# Autodesk Inventor assembly: MechanumChassis
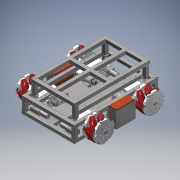
[picture p0: Inventor's stored thumbnail of the model, 180x180]
Saved by Autodesk Inventor 2018 (Build 220112000, 112)
## iProperties
Created: 2017-10-18
Part Number: MechanumChassis
Document SubType Name: Weldment
Designer: Bryce Richards
Mass: 42172.1 g
Surface Area: 44852.8 cm^2
Volume: 5448.29 cm^3
Density: 7.74044 g/cm^3
Weld Material: Steel, Mild, Welded
Author: Bryce Richards
## Documents named in this file (20)
- C:\Users\P136265\Documents\GitHub\mecanum-cad\MechanumChassis.iam
- C:\Users\P136265\Documents\GitHub\mecanum-cad\MecanumFrame2.iam
- C:\Users\P136265\Documents\GitHub\mecanum-cad\WheelShaft.ipt
- C:\Users\P136265\Documents\GitHub\mecanum-cad\Mecanum_Assembly.iam
- C:\Users\P136265\Documents\Inventor\Content Center Files\R2018\en-US\AS 1112 (2)\AS 1112 - M4  Type 5.ipt
- C:\Users\P136265\Documents\GitHub\mecanum-cad\LiftBase.ipt
- C:\Users\P136265\Documents\GitHub\mecanum-cad\BatteryBox_NP1812.ipt
- C:\Users\P136265\Documents\GitHub\mecanum-cad\NP18-12 Battery.ipt
- C:\Users\P136265\Documents\GitHub\mecanum-cad\BearingHousing.iam
- C:\Users\P136265\Documents\Inventor\Content Center Files\R2018\en-US\AS 1110\AS 1110 - M8 x 50.ipt
- C:\Users\P136265\Documents\GitHub\mecanum-cad\mount.ipt
- C:\Users\P136265\Documents\GitHub\mecanum-cad\Nema 23 Stepper Motor Bipolar L=56mm w Gear Ratio 41 Planetary Gearbox.ipt
- C:\Users\P136265\Documents\GitHub\mecanum-cad\LiftAssembly_Through.iam
- C:\Users\P136265\Documents\Inventor\Content Center Files\R2018\en-US\BS EN 24035\ISO 4035 - M20BS EN.ipt
- C:\Users\P136265\Documents\Inventor\Content Center Files\R2018\en-US\AS 1420\AS 1420 - 1973 - M4 x 12.ipt
- C:\Users\P136265\Documents\Inventor\Content Center Files\R2018\en-US\AS 1112 (2)\AS 1112 - M8  Type 8.ipt
- C:\Users\P136265\Documents\GitHub\mecanum-cad\SyncHub_Assembly.iam
- C:\Users\P136265\Documents\Inventor\Content Center Files\R2018\en-US\BS EN 24035\ISO 4035 - M12BS EN.ipt
- C:\Users\P136265\Documents\GitHub\mecanum-cad\LiftPlate.iam
- C:\Users\P136265\Documents\mecanum-cad\MechanumChassis\AIP\FEA\cayefugld.fres
## Components (91 placed, 18 different names)
1. MecanumFrame2:1 [sub-assembly] — Mate:90, Angle:5, Angle:6, Angle:7, Mate:386, Flush:32, Flush:33, Mate:486, Mate:487, Mate:488, Mate:489, Mate:494, Mate:500, Mate:501, Mate:502, Mate:503, Mate:504, Mate:594, Angle:41, Mate:607, Mate:608, Mate:641, Mate:642, Mate:643, Mate:644, Mate:645, Mate:646, Angle:49, Angle:51, Insert:1, Insert:2, Insert:3, Insert:4, Insert:5, Insert:6, Insert:7, Insert:8, Insert:9, Insert:10, Insert:11, Insert:12, Insert:13, Insert:14, Insert:15, Insert:16, Angle:52, Angle:53
2. Mecanum_Assembly:1 [sub-assembly] — Mate:617, Mate:618, Angle:44, Mate:654
3. Mecanum_Assembly:2 [sub-assembly] — Mate:613, Mate:614, Angle:43, Mate:652
4. Mecanum_Assembly:3 [sub-assembly] — Mate:621, Mate:622, Mate:650
5. Mecanum_Assembly:4 [sub-assembly] — Mate:609, Mate:610, Angle:42, Mate:648
6. LiftBase:1 — Mate:386, Flush:32, Flush:33, Mate:606, Mate:635, Mate:637, Mate:639
7. BatteryBox_NP1812:1 — Mate:459, Mate:461
8. BatteryBox_NP1812:2 — Mate:462, Mate:464
9. NP18-12 Battery:1 — Mate:459, Mate:461, Angle:45, Angle:46
10. NP18-12 Battery:2 — Mate:462, Mate:464, Angle:40, Angle:47
11. AS 1112 (2) - Metric M4  Type 5:17
12. AS 1112 (2) - Metric M4  Type 5:18
13. AS 1112 (2) - Metric M4  Type 5:19
14. AS 1112 (2) - Metric M4  Type 5:20
15. AS 1112 (2) - Metric M4  Type 5:21
16. AS 1112 (2) - Metric M4  Type 5:22
17. AS 1112 (2) - Metric M4  Type 5:23
18. AS 1112 (2) - Metric M4  Type 5:24
19. BearingHousing:1 [sub-assembly] — Mate:486, Mate:487, Mate:488, Mate:489, Mate:493, Mate:611, Mate:612, Mate:660, Mate:672, Mate:674, Mate:676, Mate:678
20. BearingHousing:2 [sub-assembly] — Mate:493, Mate:494, Mate:594, Mate:615, Mate:616, Mate:658, Mate:696, Mate:698, Mate:700, Mate:702
21. BearingHousing:3 [sub-assembly] — Mate:503, Mate:504, Mate:623, Mate:624, Mate:662, Mate:680, Mate:682, Mate:684, Mate:686
22. BearingHousing:4 [sub-assembly] — Mate:500, Mate:501, Mate:502, Mate:619, Mate:620, Mate:656, Mate:688, Mate:690, Mate:692, Mate:694
23. mount:1 — Mate:603, Mate:604, Mate:605, Mate:606
24. Nema 23 Stepper Motor Bipolar L=56mm w Gear Ratio 41 Planetary Gearbox:1 — Mate:603, Mate:604, Mate:605, Angle:40, Angle:41, Flush:34, Mate:625, Mate:711
25. LiftAssembly_Through:1 [sub-assembly] — Mate:607, Mate:608, Angle:48
26. WheelShaft:1 — Mate:621, Mate:622, Mate:623, Mate:624, Flush:37, Mate:640, Mate:649, Mate:661, Mate:709, Flush:38, Mate:715
27. WheelShaft:2 — Mate:617, Mate:618, Mate:619, Mate:620, Angle:44, Flush:36, Mate:638, Mate:653, Mate:655, Mate:708, Mate:713
28. WheelShaft:3 — Mate:613, Mate:614, Mate:615, Mate:616, Angle:43, Flush:35, Mate:636, Mate:651, Mate:657, Mate:704, Mate:717
29. WheelShaft:4 — Mate:609, Mate:610, Angle:42, Mate:611, Mate:612, Flush:34, Mate:625, Mate:647, Mate:659, Mate:712, Flush:39, Mate:719
30. mount:2 — Mate:626, Mate:627, Mate:628, Mate:637
31. mount:3 — Mate:629, Mate:630, Mate:631, Mate:639
32. mount:4 — Mate:632, Mate:633, Mate:634, Mate:635
33. Nema 23 Stepper Motor Bipolar L=56mm w Gear Ratio 41 Planetary Gearbox:2 — Mate:626, Mate:627, Mate:628, Angle:46, Flush:36, Mate:638, Mate:706
34. Nema 23 Stepper Motor Bipolar L=56mm w Gear Ratio 41 Planetary Gearbox:3 — Mate:629, Mate:630, Mate:631, Angle:47, Flush:37, Mate:640, Mate:710
35. Nema 23 Stepper Motor Bipolar L=56mm w Gear Ratio 41 Planetary Gearbox:4 — Mate:632, Mate:633, Mate:634, Angle:45, Flush:35, Mate:636, Mate:705
36. LiftAssembly_Through:2 [sub-assembly] — Mate:641, Mate:642, Angle:50, Angle:51, Mate:663, Mate:664, Mate:665, Mate:666, Mate:667, Mate:668, Mate:669, Mate:670
37. LiftAssembly_Through:3 [sub-assembly] — Mate:643, Mate:644, Angle:50, Mate:721
38. LiftAssembly_Through:4 [sub-assembly] — Mate:645, Mate:646, Angle:48, Angle:49
39. BS EN 24035 - Metric M20:1 — Mate:647, Mate:648
40. BS EN 24035 - Metric M20:2 — Mate:649, Mate:650
41. BS EN 24035 - Metric M20:3 — Mate:651, Mate:652
42. BS EN 24035 - Metric M20:4 — Mate:653, Mate:654
43. BS EN 24035 - Metric M20:5 — Mate:655, Mate:656, Mate:707
44. BS EN 24035 - Metric M20:6 — Mate:657, Mate:658, Mate:703
45. BS EN 24035 - Metric M20:7 — Mate:659, Mate:660
46. BS EN 24035 - Metric M20:8 — Mate:661, Mate:662
47. AS 1110 - Metric M8 x 50:1 — Insert:1, Mate:697
48. AS 1110 - Metric M8 x 50:2 — Insert:2, Mate:699
49. AS 1110 - Metric M8 x 50:3 — Insert:3, Mate:693
50. AS 1110 - Metric M8 x 50:4 — Insert:4, Mate:691
51. AS 1110 - Metric M8 x 50:5 — Insert:5, Mate:695
52. AS 1110 - Metric M8 x 50:6 — Insert:6, Mate:701
53. AS 1110 - Metric M8 x 50:7 — Insert:7, Mate:687
54. AS 1110 - Metric M8 x 50:8 — Insert:8, Mate:689
55. AS 1110 - Metric M8 x 50:9 — Insert:9, Mate:675
56. AS 1110 - Metric M8 x 50:10 — Insert:10, Mate:677
57. AS 1110 - Metric M8 x 50:11 — Insert:11, Mate:685
58. AS 1110 - Metric M8 x 50:12 — Insert:12, Mate:683
59. AS 1110 - Metric M8 x 50:13 — Insert:13, Mate:671
60. AS 1110 - Metric M8 x 50:14 — Insert:14, Mate:673
61. AS 1110 - Metric M8 x 50:15 — Insert:15, Mate:679
62. AS 1110 - Metric M8 x 50:16 — Insert:16, Mate:681
63. AS 1420 - Metric M4 x 12:1 — Mate:663, Mate:664
64. AS 1420 - Metric M4 x 12:2 — Mate:665, Mate:666
65. AS 1420 - Metric M4 x 12:3 — Mate:667, Mate:668
66. AS 1420 - Metric M4 x 12:4 — Mate:669, Mate:670
67. AS 1112 (2) - Metric M8  Type 8:1 — Mate:671, Mate:672
68. AS 1112 (2) - Metric M8  Type 8:2 — Mate:673, Mate:674
69. AS 1112 (2) - Metric M8  Type 8:3 — Mate:675, Mate:676
70. AS 1112 (2) - Metric M8  Type 8:4 — Mate:677, Mate:678
71. AS 1112 (2) - Metric M8  Type 8:5 — Mate:679, Mate:680
72. AS 1112 (2) - Metric M8  Type 8:6 — Mate:681, Mate:682
73. AS 1112 (2) - Metric M8  Type 8:7 — Mate:683, Mate:684
74. AS 1112 (2) - Metric M8  Type 8:8 — Mate:685, Mate:686
75. AS 1112 (2) - Metric M8  Type 8:9 — Mate:687, Mate:688
76. AS 1112 (2) - Metric M8  Type 8:10 — Mate:689, Mate:690
77. AS 1112 (2) - Metric M8  Type 8:11 — Mate:691, Mate:692
78. AS 1112 (2) - Metric M8  Type 8:12 — Mate:693, Mate:694
79. AS 1112 (2) - Metric M8  Type 8:13 — Mate:695, Mate:696
80. AS 1112 (2) - Metric M8  Type 8:14 — Mate:697, Mate:698
81. AS 1112 (2) - Metric M8  Type 8:15 — Mate:699, Mate:700
82. AS 1112 (2) - Metric M8  Type 8:16 — Mate:701, Mate:702
83. SyncHub_Assembly:1 [sub-assembly] — Mate:703, Mate:704, Mate:705, Mate:718
84. SyncHub_Assembly:2 [sub-assembly] — Mate:711, Mate:712, Flush:39, Mate:720
85. SyncHub_Assembly:3 [sub-assembly] — Mate:706, Mate:707, Mate:708, Mate:714
86. SyncHub_Assembly:4 [sub-assembly] — Mate:709, Mate:710, Flush:38, Mate:716
87. BS EN 24035 - Metric M12:1 — Mate:713, Mate:714
88. BS EN 24035 - Metric M12:2 — Mate:715, Mate:716
89. BS EN 24035 - Metric M12:3 — Mate:717, Mate:718
90. BS EN 24035 - Metric M12:4 — Mate:719, Mate:720
91. LiftPlate:1 [sub-assembly] — Angle:52, Angle:53, Mate:721
## Relationships (178: Mate 137, Angle 17, Insert 16, Flush 8)
- Mate:90: MecanumFrame2:1
- Angle:5 (0 deg): MecanumFrame2:1
- Angle:6 (0 deg): MecanumFrame2:1
- Angle:7 (0 deg): MecanumFrame2:1
- Mate:386: MecanumFrame2:1 ↔ LiftBase:1
- Flush:32 (2.5 mm): MecanumFrame2:1 ↔ LiftBase:1
- Flush:33 (2.5 mm): MecanumFrame2:1 ↔ LiftBase:1
- Mate:459: BatteryBox_NP1812:1 ↔ NP18-12 Battery:1
- Mate:461 (2 mm): BatteryBox_NP1812:1 ↔ NP18-12 Battery:1
- Mate:462: BatteryBox_NP1812:2 ↔ NP18-12 Battery:2
- Mate:464 (2 mm): BatteryBox_NP1812:2 ↔ NP18-12 Battery:2
- Mate:486: MecanumFrame2:1 ↔ BearingHousing:1
- Mate:487: MecanumFrame2:1 ↔ BearingHousing:1
- Mate:488: MecanumFrame2:1 ↔ BearingHousing:1
- Mate:489: MecanumFrame2:1 ↔ BearingHousing:1
- Mate:493: BearingHousing:1 ↔ BearingHousing:2
- Mate:494: MecanumFrame2:1 ↔ BearingHousing:2
- Mate:500: MecanumFrame2:1 ↔ BearingHousing:4
- Mate:501: MecanumFrame2:1 ↔ BearingHousing:4
- Mate:502: MecanumFrame2:1 ↔ BearingHousing:4
- Mate:503: MecanumFrame2:1 ↔ BearingHousing:3
- Mate:504: MecanumFrame2:1 ↔ BearingHousing:3
- Mate:594: MecanumFrame2:1 ↔ BearingHousing:2
- Mate:603: mount:1 ↔ Nema 23 Stepper Motor Bipolar L=56mm w Gear Ratio 41 Planetary Gearbox:1
- Mate:604: mount:1 ↔ Nema 23 Stepper Motor Bipolar L=56mm w Gear Ratio 41 Planetary Gearbox:1
- Mate:605: mount:1 ↔ Nema 23 Stepper Motor Bipolar L=56mm w Gear Ratio 41 Planetary Gearbox:1
- Mate:606: LiftBase:1 ↔ mount:1
- Angle:40 (180 deg): NP18-12 Battery:2 ↔ Nema 23 Stepper Motor Bipolar L=56mm w Gear Ratio 41 Planetary Gearbox:1
- Angle:41 (0 deg): MecanumFrame2:1 ↔ Nema 23 Stepper Motor Bipolar L=56mm w Gear Ratio 41 Planetary Gearbox:1
- Mate:607: MecanumFrame2:1 ↔ LiftAssembly_Through:1
- Mate:608: MecanumFrame2:1 ↔ LiftAssembly_Through:1
- Mate:609: Mecanum_Assembly:4 ↔ WheelShaft:4
- Mate:610: Mecanum_Assembly:4 ↔ WheelShaft:4
- Angle:42 (0 deg): Mecanum_Assembly:4 ↔ WheelShaft:4
- Mate:611: BearingHousing:1 ↔ WheelShaft:4
- Mate:612: BearingHousing:1 ↔ WheelShaft:4
- Flush:34 (10 mm): Nema 23 Stepper Motor Bipolar L=56mm w Gear Ratio 41 Planetary Gearbox:1 ↔ WheelShaft:4
- Mate:613: Mecanum_Assembly:2 ↔ WheelShaft:3
- Mate:614: Mecanum_Assembly:2 ↔ WheelShaft:3
- Mate:615: BearingHousing:2 ↔ WheelShaft:3
- Mate:616: BearingHousing:2 ↔ WheelShaft:3
- Angle:43 (0 deg): Mecanum_Assembly:2 ↔ WheelShaft:3
- Mate:617: Mecanum_Assembly:1 ↔ WheelShaft:2
- Mate:618: Mecanum_Assembly:1 ↔ WheelShaft:2
- Mate:619: BearingHousing:4 ↔ WheelShaft:2
- Mate:620: BearingHousing:4 ↔ WheelShaft:2
- Angle:44 (0 deg): Mecanum_Assembly:1 ↔ WheelShaft:2
- Mate:621: Mecanum_Assembly:3 ↔ WheelShaft:1
- Mate:622: Mecanum_Assembly:3 ↔ WheelShaft:1
- Mate:623: BearingHousing:3 ↔ WheelShaft:1
- Mate:624: BearingHousing:3 ↔ WheelShaft:1
- Mate:625 (107.5 mm): Nema 23 Stepper Motor Bipolar L=56mm w Gear Ratio 41 Planetary Gearbox:1 ↔ WheelShaft:4
- Mate:626: mount:2 ↔ Nema 23 Stepper Motor Bipolar L=56mm w Gear Ratio 41 Planetary Gearbox:2
- Mate:627: mount:2 ↔ Nema 23 Stepper Motor Bipolar L=56mm w Gear Ratio 41 Planetary Gearbox:2
- Mate:628: mount:2 ↔ Nema 23 Stepper Motor Bipolar L=56mm w Gear Ratio 41 Planetary Gearbox:2
- Mate:629: mount:3 ↔ Nema 23 Stepper Motor Bipolar L=56mm w Gear Ratio 41 Planetary Gearbox:3
- Mate:630: mount:3 ↔ Nema 23 Stepper Motor Bipolar L=56mm w Gear Ratio 41 Planetary Gearbox:3
- Mate:631: mount:3 ↔ Nema 23 Stepper Motor Bipolar L=56mm w Gear Ratio 41 Planetary Gearbox:3
- Mate:632: mount:4 ↔ Nema 23 Stepper Motor Bipolar L=56mm w Gear Ratio 41 Planetary Gearbox:4
- Mate:633: mount:4 ↔ Nema 23 Stepper Motor Bipolar L=56mm w Gear Ratio 41 Planetary Gearbox:4
- Mate:634: mount:4 ↔ Nema 23 Stepper Motor Bipolar L=56mm w Gear Ratio 41 Planetary Gearbox:4
- Mate:635: LiftBase:1 ↔ mount:4
- Angle:45 (0 deg): NP18-12 Battery:1 ↔ Nema 23 Stepper Motor Bipolar L=56mm w Gear Ratio 41 Planetary Gearbox:4
- Flush:35 (10 mm): WheelShaft:3 ↔ Nema 23 Stepper Motor Bipolar L=56mm w Gear Ratio 41 Planetary Gearbox:4
- Mate:636 (107.5 mm): WheelShaft:3 ↔ Nema 23 Stepper Motor Bipolar L=56mm w Gear Ratio 41 Planetary Gearbox:4
- Mate:637: LiftBase:1 ↔ mount:2
- Angle:46 (0 deg): NP18-12 Battery:1 ↔ Nema 23 Stepper Motor Bipolar L=56mm w Gear Ratio 41 Planetary Gearbox:2
- Flush:36 (10 mm): WheelShaft:2 ↔ Nema 23 Stepper Motor Bipolar L=56mm w Gear Ratio 41 Planetary Gearbox:2
- Mate:638 (107.5 mm): WheelShaft:2 ↔ Nema 23 Stepper Motor Bipolar L=56mm w Gear Ratio 41 Planetary Gearbox:2
- Angle:47 (0 deg): NP18-12 Battery:2 ↔ Nema 23 Stepper Motor Bipolar L=56mm w Gear Ratio 41 Planetary Gearbox:3
- Mate:639: LiftBase:1 ↔ mount:3
- Flush:37 (10 mm): WheelShaft:1 ↔ Nema 23 Stepper Motor Bipolar L=56mm w Gear Ratio 41 Planetary Gearbox:3
- Mate:640 (107.5 mm): WheelShaft:1 ↔ Nema 23 Stepper Motor Bipolar L=56mm w Gear Ratio 41 Planetary Gearbox:3
- Mate:641: MecanumFrame2:1 ↔ LiftAssembly_Through:2
- Mate:642: MecanumFrame2:1 ↔ LiftAssembly_Through:2
- Mate:643: MecanumFrame2:1 ↔ LiftAssembly_Through:3
- Mate:644: MecanumFrame2:1 ↔ LiftAssembly_Through:3
- Mate:645: MecanumFrame2:1 ↔ LiftAssembly_Through:4
- Mate:646: MecanumFrame2:1 ↔ LiftAssembly_Through:4
- Angle:48 (0 deg): LiftAssembly_Through:1 ↔ LiftAssembly_Through:4
- Angle:49 (0 deg): MecanumFrame2:1 ↔ LiftAssembly_Through:4
- Angle:50 (0 deg): LiftAssembly_Through:2 ↔ LiftAssembly_Through:3
- Angle:51 (0 deg): MecanumFrame2:1 ↔ LiftAssembly_Through:2
- Mate:647: WheelShaft:4 ↔ BS EN 24035 - Metric M20:1
- Mate:648: Mecanum_Assembly:4 ↔ BS EN 24035 - Metric M20:1
- Mate:649: WheelShaft:1 ↔ BS EN 24035 - Metric M20:2
- Mate:650: Mecanum_Assembly:3 ↔ BS EN 24035 - Metric M20:2
- Mate:651: WheelShaft:3 ↔ BS EN 24035 - Metric M20:3
- Mate:652: Mecanum_Assembly:2 ↔ BS EN 24035 - Metric M20:3
- Mate:653: WheelShaft:2 ↔ BS EN 24035 - Metric M20:4
- Mate:654: Mecanum_Assembly:1 ↔ BS EN 24035 - Metric M20:4
- Mate:655: WheelShaft:2 ↔ BS EN 24035 - Metric M20:5
- Mate:656: BearingHousing:4 ↔ BS EN 24035 - Metric M20:5
- Mate:657: WheelShaft:3 ↔ BS EN 24035 - Metric M20:6
- Mate:658: BearingHousing:2 ↔ BS EN 24035 - Metric M20:6
- Mate:659: WheelShaft:4 ↔ BS EN 24035 - Metric M20:7
- Mate:660: BearingHousing:1 ↔ BS EN 24035 - Metric M20:7
- Mate:661: WheelShaft:1 ↔ BS EN 24035 - Metric M20:8
- Mate:662: BearingHousing:3 ↔ BS EN 24035 - Metric M20:8
- Insert:1: MecanumFrame2:1 ↔ AS 1110 - Metric M8 x 50:1
- Insert:2: MecanumFrame2:1 ↔ AS 1110 - Metric M8 x 50:2
- Insert:3: MecanumFrame2:1 ↔ AS 1110 - Metric M8 x 50:3
- Insert:4: MecanumFrame2:1 ↔ AS 1110 - Metric M8 x 50:4
- Insert:5: MecanumFrame2:1 ↔ AS 1110 - Metric M8 x 50:5
- Insert:6: MecanumFrame2:1 ↔ AS 1110 - Metric M8 x 50:6
- Insert:7: MecanumFrame2:1 ↔ AS 1110 - Metric M8 x 50:7
- Insert:8: MecanumFrame2:1 ↔ AS 1110 - Metric M8 x 50:8
- Insert:9: MecanumFrame2:1 ↔ AS 1110 - Metric M8 x 50:9
- Insert:10: MecanumFrame2:1 ↔ AS 1110 - Metric M8 x 50:10
- Insert:11: MecanumFrame2:1 ↔ AS 1110 - Metric M8 x 50:11
- Insert:12: MecanumFrame2:1 ↔ AS 1110 - Metric M8 x 50:12
- Insert:13: MecanumFrame2:1 ↔ AS 1110 - Metric M8 x 50:13
- Insert:14: MecanumFrame2:1 ↔ AS 1110 - Metric M8 x 50:14
- Insert:15: MecanumFrame2:1 ↔ AS 1110 - Metric M8 x 50:15
- Insert:16: MecanumFrame2:1 ↔ AS 1110 - Metric M8 x 50:16
- Mate:663: LiftAssembly_Through:2 ↔ AS 1420 - Metric M4 x 12:1
- Mate:664: LiftAssembly_Through:2 ↔ AS 1420 - Metric M4 x 12:1
- Mate:665: LiftAssembly_Through:2 ↔ AS 1420 - Metric M4 x 12:2
- Mate:666: LiftAssembly_Through:2 ↔ AS 1420 - Metric M4 x 12:2
- Mate:667: LiftAssembly_Through:2 ↔ AS 1420 - Metric M4 x 12:3
- Mate:668: LiftAssembly_Through:2 ↔ AS 1420 - Metric M4 x 12:3
- Mate:669: LiftAssembly_Through:2 ↔ AS 1420 - Metric M4 x 12:4
- Mate:670: LiftAssembly_Through:2 ↔ AS 1420 - Metric M4 x 12:4
- Mate:671: AS 1110 - Metric M8 x 50:13 ↔ AS 1112 (2) - Metric M8  Type 8:1
- Mate:672: BearingHousing:1 ↔ AS 1112 (2) - Metric M8  Type 8:1
- Mate:673: AS 1110 - Metric M8 x 50:14 ↔ AS 1112 (2) - Metric M8  Type 8:2
- Mate:674: BearingHousing:1 ↔ AS 1112 (2) - Metric M8  Type 8:2
- Mate:675: AS 1110 - Metric M8 x 50:9 ↔ AS 1112 (2) - Metric M8  Type 8:3
- Mate:676: BearingHousing:1 ↔ AS 1112 (2) - Metric M8  Type 8:3
- Mate:677: AS 1110 - Metric M8 x 50:10 ↔ AS 1112 (2) - Metric M8  Type 8:4
- Mate:678: BearingHousing:1 ↔ AS 1112 (2) - Metric M8  Type 8:4
- Mate:679: AS 1110 - Metric M8 x 50:15 ↔ AS 1112 (2) - Metric M8  Type 8:5
- Mate:680: BearingHousing:3 ↔ AS 1112 (2) - Metric M8  Type 8:5
- Mate:681: AS 1110 - Metric M8 x 50:16 ↔ AS 1112 (2) - Metric M8  Type 8:6
- Mate:682: BearingHousing:3 ↔ AS 1112 (2) - Metric M8  Type 8:6
- Mate:683: AS 1110 - Metric M8 x 50:12 ↔ AS 1112 (2) - Metric M8  Type 8:7
- Mate:684: BearingHousing:3 ↔ AS 1112 (2) - Metric M8  Type 8:7
- Mate:685: AS 1110 - Metric M8 x 50:11 ↔ AS 1112 (2) - Metric M8  Type 8:8
- Mate:686: BearingHousing:3 ↔ AS 1112 (2) - Metric M8  Type 8:8
- Mate:687: AS 1110 - Metric M8 x 50:7 ↔ AS 1112 (2) - Metric M8  Type 8:9
- Mate:688: BearingHousing:4 ↔ AS 1112 (2) - Metric M8  Type 8:9
- Mate:689: AS 1110 - Metric M8 x 50:8 ↔ AS 1112 (2) - Metric M8  Type 8:10
- Mate:690: BearingHousing:4 ↔ AS 1112 (2) - Metric M8  Type 8:10
- Mate:691: AS 1110 - Metric M8 x 50:4 ↔ AS 1112 (2) - Metric M8  Type 8:11
- Mate:692: BearingHousing:4 ↔ AS 1112 (2) - Metric M8  Type 8:11
- Mate:693: AS 1110 - Metric M8 x 50:3 ↔ AS 1112 (2) - Metric M8  Type 8:12
- Mate:694: BearingHousing:4 ↔ AS 1112 (2) - Metric M8  Type 8:12
- Mate:695: AS 1110 - Metric M8 x 50:5 ↔ AS 1112 (2) - Metric M8  Type 8:13
- Mate:696: BearingHousing:2 ↔ AS 1112 (2) - Metric M8  Type 8:13
- Mate:697: AS 1110 - Metric M8 x 50:1 ↔ AS 1112 (2) - Metric M8  Type 8:14
- Mate:698: BearingHousing:2 ↔ AS 1112 (2) - Metric M8  Type 8:14
- Mate:699: AS 1110 - Metric M8 x 50:2 ↔ AS 1112 (2) - Metric M8  Type 8:15
- Mate:700: BearingHousing:2 ↔ AS 1112 (2) - Metric M8  Type 8:15
- Mate:701: AS 1110 - Metric M8 x 50:6 ↔ AS 1112 (2) - Metric M8  Type 8:16
- Mate:702: BearingHousing:2 ↔ AS 1112 (2) - Metric M8  Type 8:16
- Mate:703: BS EN 24035 - Metric M20:6 ↔ SyncHub_Assembly:1
- Mate:704: WheelShaft:3 ↔ SyncHub_Assembly:1
- Mate:705: Nema 23 Stepper Motor Bipolar L=56mm w Gear Ratio 41 Planetary Gearbox:4 ↔ SyncHub_Assembly:1
- Mate:706: Nema 23 Stepper Motor Bipolar L=56mm w Gear Ratio 41 Planetary Gearbox:2 ↔ SyncHub_Assembly:3
- Mate:707: BS EN 24035 - Metric M20:5 ↔ SyncHub_Assembly:3
- Mate:708: WheelShaft:2 ↔ SyncHub_Assembly:3
- Mate:709: WheelShaft:1 ↔ SyncHub_Assembly:4
- Mate:710: Nema 23 Stepper Motor Bipolar L=56mm w Gear Ratio 41 Planetary Gearbox:3 ↔ SyncHub_Assembly:4
- Flush:38 (-10 mm): WheelShaft:1 ↔ SyncHub_Assembly:4
- Mate:711: Nema 23 Stepper Motor Bipolar L=56mm w Gear Ratio 41 Planetary Gearbox:1 ↔ SyncHub_Assembly:2
- Mate:712: WheelShaft:4 ↔ SyncHub_Assembly:2
- Flush:39 (10 mm): WheelShaft:4 ↔ SyncHub_Assembly:2
- Mate:713: WheelShaft:2 ↔ BS EN 24035 - Metric M12:1
- Mate:714: SyncHub_Assembly:3 ↔ BS EN 24035 - Metric M12:1
- Mate:715: WheelShaft:1 ↔ BS EN 24035 - Metric M12:2
- Mate:716: SyncHub_Assembly:4 ↔ BS EN 24035 - Metric M12:2
- Mate:717: WheelShaft:3 ↔ BS EN 24035 - Metric M12:3
- Mate:718: SyncHub_Assembly:1 ↔ BS EN 24035 - Metric M12:3
- Mate:719: WheelShaft:4 ↔ BS EN 24035 - Metric M12:4
- Mate:720: SyncHub_Assembly:2 ↔ BS EN 24035 - Metric M12:4
- Angle:52 (0 deg): MecanumFrame2:1 ↔ LiftPlate:1
- Angle:53 (0 deg): MecanumFrame2:1 ↔ LiftPlate:1
- Mate:721: LiftAssembly_Through:3 ↔ LiftPlate:1
## Named parameters: sa_0 = 0, sa_1 = -3.88819e-08, sa_2 = 1e+06
note: some values were not read from the file. Shown as the stored number, unit unknown: "sa_0", "sa_1", "sa_2".
